# Autodesk Inventor assembly: SoccerField_KidSize
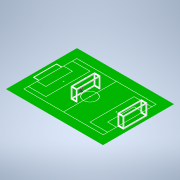
[picture p0: Inventor's stored thumbnail of the model, 180x180]
Saved by Autodesk Inventor 2022 (Build 260153000, 153)
## iProperties
Created: 2022-10-30
Part Number: SoccerField_KidSize
Document SubType Name: Assembly
Designer: Masato Kubotera
Author: Masato Kubotera
## Documents named in this file (4)
- C:\Users\MasatoKubotera\Desktop\RoboCupHumanoidLeagueSoccerField\SoccerField_KidSize.iam
- C:\Users\MasatoKubotera\Desktop\RoboCupHumanoidLeagueSoccerField\Goal.ipt
- C:\Users\MasatoKubotera\Desktop\RoboCupHumanoidLeagueSoccerField\SoccerField_KidSize.ipt
- C:\Users\MasatoKubotera\Desktop\SUSTAINA-OP\Body.iam
## Components (4 placed, 3 different names)
1. SoccerField_KidSize:1 — フラッシュ:1, フラッシュ:2, フラッシュ:3, フラッシュ:4, フラッシュ:5, メイト:1
2. Goal:1 — フラッシュ:4, フラッシュ:5, メイト:1
3. Goal:2
4. Body:1 [sub-assembly]
## Relationships (6: Flush 5, Mate 1)
- フラッシュ:1 [Flush]: SoccerField_KidSize:1
- フラッシュ:2 [Flush]: SoccerField_KidSize:1
- フラッシュ:3 [Flush]: SoccerField_KidSize:1
- フラッシュ:4 [Flush]: SoccerField_KidSize:1 ↔ Goal:1
- フラッシュ:5 [Flush]: SoccerField_KidSize:1 ↔ Goal:1
- メイト:1 [Mate]: SoccerField_KidSize:1 ↔ Goal:1
